# Autodesk Inventor assembly: ENSAMBLE GENERAL ACH-40L-2020-V
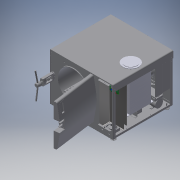
[picture p0: Inventor's stored thumbnail of the model, 180x180]
Saved by Autodesk Inventor 2017 (Build 210142000, 142)
## iProperties
Created: 2020-09-24
Part Number: ENSAMBLE GENERAL ACH-40L-2020-V
Description: STEP AP203
Document SubType Name: Assembly
Designer: USUARIO
Title: ENSAMBLE GENERAL ACH-40L-2020-V.STEP
Revision Number: ANY
Sending System: SolidWorks 2013
Preprocessor: SwSTEP 2.0
## Documents named in this file (42)
- D:\Laboratorio\Autoclave\Autoclave Horizontal\Sin Precamara\2020\Autoclave 40L con Vacio Insulab #0045883XX OP2020292\ENSAMBLE GENERAL ACH-40L-2020-V.iam
- D:\Laboratorio\Autoclave\Autoclave Horizontal\Sin Precamara\2020\Autoclave 40L con Vacio Insulab #0045883XX OP2020292\CUBIERTA FRONTAL ACH-40L-2020-V.ipt
- D:\Laboratorio\Autoclave\Autoclave Horizontal\Sin Precamara\2020\Autoclave 40L con Vacio Insulab #0045883XX OP2020292\BASE MUEBLE ACH-40L-2020-V.ipt
- D:\Laboratorio\Autoclave\Autoclave Horizontal\Sin Precamara\2020\Autoclave 40L con Vacio Insulab #0045883XX OP2020292\MARCO POSTERIOR ACH-40L-2020-V.ipt
- D:\Laboratorio\Autoclave\Autoclave Horizontal\Sin Precamara\2020\Autoclave 40L con Vacio Insulab #0045883XX OP2020292\ENSAMBLE TANQUE ACH-40L-2020-V.iam
- D:\Laboratorio\Autoclave\Autoclave Horizontal\Sin Precamara\2020\Autoclave 40L con Vacio Insulab #0045883XX OP2020292\ENSAMBLE PANEL FRONTAL ACH-40L-2020-V.iam
- D:\Laboratorio\Autoclave\Autoclave Horizontal\Sin Precamara\2020\Autoclave 40L con Vacio Insulab #0045883XX OP2020292\ENSAMBLE PUERTA ACH-40L-2020-V.iam
- D:\Laboratorio\Autoclave\Autoclave Horizontal\Sin Precamara\2020\Autoclave 40L con Vacio Insulab #0045883XX OP2020292\CAJA CONEXIONES ESPINAS ACH-40L-2020-V.ipt
- D:\Laboratorio\Autoclave\Autoclave Horizontal\Sin Precamara\2020\Autoclave 40L con Vacio Insulab #0045883XX OP2020292\PG-13,5.ipt
- D:\Laboratorio\Autoclave\Autoclave Horizontal\Sin Precamara\2020\Autoclave 40L con Vacio Insulab #0045883XX OP2020292\CAJA CONEXIONES ACH-40L-2020-V.ipt
- D:\Laboratorio\Autoclave\Autoclave Horizontal\Sin Precamara\2020\Autoclave 40L con Vacio Insulab #0045883XX OP2020292\REFUERZO INTERIOR ACH-40L-2020-V.ipt
- D:\Laboratorio\Autoclave\Autoclave Horizontal\Sin Precamara\2020\Autoclave 40L con Vacio Insulab #0045883XX OP2020292\VENTILADOR 9X9.ipt
- D:\Laboratorio\Autoclave\Autoclave Horizontal\Sin Precamara\2020\Autoclave 40L con Vacio Insulab #0045883XX OP2020292\ENSAMBLE GENERAL CIERRE JP2019-TTNR.iam
- D:\Laboratorio\Autoclave\Autoclave Horizontal\Sin Precamara\2020\Autoclave 40L con Vacio Insulab #0045883XX OP2020292\PIN CIERRE JP2019-TTNR.ipt
- D:\Laboratorio\Autoclave\Autoclave Horizontal\Sin Precamara\2020\Autoclave 40L con Vacio Insulab #0045883XX OP2020292\PIN BISAGRA JP2019-TTNR.ipt
- D:\Laboratorio\Autoclave\Autoclave Horizontal\Sin Precamara\2020\Autoclave 40L con Vacio Insulab #0045883XX OP2020292\PIVOTE CIERRE JP2019-TTNR.ipt
- D:\Laboratorio\Autoclave\Autoclave Horizontal\Sin Precamara\2020\Autoclave 40L con Vacio Insulab #0045883XX OP2020292\ENSAMBLE TAPA ACH-40L-2020-V.iam
- D:\Laboratorio\Autoclave\Autoclave Horizontal\Sin Precamara\2020\Autoclave 40L con Vacio Insulab #0045883XX OP2020292\ENSAMBLE RESERVORIO ACH-40L-2020-V.iam
- D:\Laboratorio\Autoclave\Autoclave Horizontal\Sin Precamara\2020\Autoclave 40L con Vacio Insulab #0045883XX OP2020292\CONTRATAPA SUPERIOR ACH-40L-2020-V.ipt
- D:\Laboratorio\Autoclave\Autoclave Horizontal\Sin Precamara\2020\Autoclave 40L con Vacio Insulab #0045883XX OP2020292\BANDEJA INTERIOR ACH-40L-2020-V.ipt
- D:\Laboratorio\Autoclave\Autoclave Horizontal\Sin Precamara\2020\Autoclave 40L con Vacio Insulab #0045883XX OP2020292\BOMBA DE VACIO THOMAS 2107CA20.ipt
- D:\Laboratorio\Autoclave\Autoclave Horizontal\Sin Precamara\2020\Autoclave 40L con Vacio Insulab #0045883XX OP2020292\CALDERIN ACH-40L-2020-V.ipt
- D:\Laboratorio\Autoclave\Autoclave Horizontal\Sin Precamara\2020\Autoclave 40L con Vacio Insulab #0045883XX OP2020292\CONTRATAPA INFERIOR ACH-40L-2020-V.ipt
- D:\Laboratorio\Autoclave\Autoclave Horizontal\Sin Precamara\2020\Autoclave 40L con Vacio Insulab #0045883XX OP2020292\CUBIERTA SUPERIOR ACH-40L-2020-V.ipt
- D:\Laboratorio\Autoclave\Autoclave Horizontal\Sin Precamara\2020\Autoclave 40L con Vacio Insulab #0045883XX OP2020292\CUBIERTA LATERAL ACH-40L-2020-V.ipt
- D:\Laboratorio\Autoclave\Autoclave Horizontal\Sin Precamara\2020\Autoclave 40L con Vacio Insulab #0045883XX OP2020292\ENSAMBLE RADIADOR ACH-40L-2020-V.iam
- D:\Laboratorio\Autoclave\Autoclave Horizontal\Sin Precamara\2020\Autoclave 40L con Vacio Insulab #0045883XX OP2020292\CUBIERTA LATERAL DERECHA ACH-40L-2020-V.ipt
- D:\Laboratorio\Autoclave\Autoclave Horizontal\Sin Precamara\2020\Autoclave 40L con Vacio Insulab #0045883XX OP2020292\CUBIERTA POSTERIOR ACH-40L-2020-V.ipt
- D:\Laboratorio\Autoclave\Autoclave Horizontal\Sin Precamara\2020\Autoclave 40L con Vacio Insulab #0045883XX OP2020292\ULKA EX5.ipt
- D:\Laboratorio\Autoclave\Autoclave Horizontal\Sin Precamara\2020\Autoclave 40L con Vacio Insulab #0045883XX OP2020292\DANFOSS EV215B.ipt
- D:\Laboratorio\Autoclave\Autoclave Horizontal\Sin Precamara\2020\Autoclave 40L con Vacio Insulab #0045883XX OP2020292\SOPORTE BOMBA AGUA ACH-40L-2020-V.ipt
- D:\Laboratorio\Autoclave\Autoclave Horizontal\Sin Precamara\2020\Autoclave 40L con Vacio Insulab #0045883XX OP2020292\SOPORTE VALVULAS ACH-40L-2020-V.ipt
- D:\Laboratorio\Autoclave\Autoclave Horizontal\Sin Precamara\2020\Autoclave 40L con Vacio Insulab #0045883XX OP2020292\PATA 5-16.ipt
- D:\Laboratorio\Autoclave\Autoclave Horizontal\Sin Precamara\2020\Autoclave 40L con Vacio Insulab #0045883XX OP2020292\VALVULA DE BOLA GENEBRE MH 3097-02 CW617N.ipt
- D:\Laboratorio\Autoclave\Autoclave Horizontal\Sin Precamara\2020\Autoclave 40L con Vacio Insulab #0045883XX OP2020292\ESPINAS DE PESCADO ACV-ACH.ipt
- D:\Laboratorio\Autoclave\Autoclave Horizontal\Sin Precamara\2020\Autoclave 40L con Vacio Insulab #0045883XX OP2020292\DERIVACION TANQUE ACH-40L-2020-V.ipt
- D:\Laboratorio\Autoclave\Autoclave Horizontal\Sin Precamara\2020\Autoclave 40L con Vacio Insulab #0045883XX OP2020292\TEE VALVULAS ACH-40L-2020-V.ipt
- D:\Laboratorio\Autoclave\Autoclave Horizontal\Sin Precamara\2020\Autoclave 40L con Vacio Insulab #0045883XX OP2020292\RESISTENCIA INTERIOR ACH-40L-2020-V.ipt
- D:\Laboratorio\Autoclave\Autoclave Horizontal\Sin Precamara\2020\Autoclave 40L con Vacio Insulab #0045883XX OP2020292\RESISTENCIA SECADO ACH-40L-2020-V.ipt
- D:\Laboratorio\Autoclave\Autoclave Horizontal\Sin Precamara\2020\Autoclave 40L con Vacio Insulab #0045883XX OP2020292\DEFLECTOR ACH-40L-2020-V.ipt
- D:\Laboratorio\Autoclave\Autoclave Horizontal\Sin Precamara\2020\Autoclave 40L con Vacio Insulab #0045883XX OP2020292\ACOPLE DEFLECTOR ACH-40L-2020-V.ipt
- D:\Laboratorio\Autoclave\Autoclave Horizontal\Sin Precamara\2020\Autoclave 40L con Vacio Insulab #0045883XX OP2020292\Schematic\Nextion Control SM\NextionControlV3.iam
## Components (52 placed, 52 different names)
1. CUBIERTA FRONTAL ACH-40L-2020-V_1
2. BASE MUEBLE ACH-40L-2020-V_2
3. MARCO POSTERIOR ACH-40L-2020-V_3
4. ENSAMBLE TANQUE ACH-40L-2020-V_4 [sub-assembly]
5. ENSAMBLE PANEL FRONTAL ACH-40L-2020-V_5 [sub-assembly]
6. ENSAMBLE PUERTA ACH-40L-2020-V_6 [sub-assembly]
7. CAJA CONEXIONES ESPINAS ACH-40L-2020-V_7
8. PG-13,5_8
9. CAJA CONEXIONES ACH-40L-2020-V_9 — Mate:1, Mate:2
10. REFUERZO INTERIOR ACH-40L-2020-V_10
11. REFUERZO INTERIOR ACH-40L-2020-V_11
12. VENTILADOR 9X9_12
13. ENSAMBLE GENERAL CIERRE JP2019-TTNR_13 [sub-assembly]
14. PIN CIERRE JP2019-TTNR_14
15. PIN BISAGRA JP2019-TTNR_15
16. PIN BISAGRA JP2019-TTNR_16
17. PIVOTE CIERRE JP2019-TTNR_17
18. ENSAMBLE TAPA ACH-40L-2020-V_18 [sub-assembly]
19. ENSAMBLE RESERVORIO ACH-40L-2020-V_19 [sub-assembly]
20. CONTRATAPA SUPERIOR ACH-40L-2020-V_20
21. BANDEJA INTERIOR ACH-40L-2020-V_21
22. BOMBA DE VACIO THOMAS 2107CA20_22
23. CALDERIN ACH-40L-2020-V_23
24. CONTRATAPA INFERIOR ACH-40L-2020-V_24
25. CUBIERTA SUPERIOR ACH-40L-2020-V_25
26. CUBIERTA LATERAL ACH-40L-2020-V_26
27. ENSAMBLE RADIADOR ACH-40L-2020-V_27 [sub-assembly]
28. CUBIERTA LATERAL DERECHA ACH-40L-2020-V_28
29. CUBIERTA POSTERIOR ACH-40L-2020-V_29
30. ULKA EX5_30
31. DANFOSS EV215B_31
32. SOPORTE BOMBA AGUA ACH-40L-2020-V_32
33. SOPORTE VALVULAS ACH-40L-2020-V_33
34. DANFOSS EV215B_34
35. DANFOSS EV215B_35
36. DANFOSS EV215B_36
37. DANFOSS EV215B_37
38. DANFOSS EV215B_38
39. PATA 5-16_39
40. PATA 5-16_40
41. PATA 5-16_41
42. PATA 5-16_42
43. PG-13,5_43
44. VALVULA DE BOLA GENEBRE MH 3097-02 CW617N_44
45. ESPINAS DE PESCADO ACV-ACH_45
46. DERIVACION TANQUE ACH-40L-2020-V_46
47. TEE VALVULAS ACH-40L-2020-V_47
48. RESISTENCIA INTERIOR ACH-40L-2020-V_48
49. RESISTENCIA SECADO ACH-40L-2020-V_49
50. DEFLECTOR ACH-40L-2020-V_50
51. ACOPLE DEFLECTOR ACH-40L-2020-V_51
52. NextionControlV3:1 [sub-assembly] — Mate:1, Mate:2
## Relationships (2: Mate 2)
- Mate:1 (10 mm): CAJA CONEXIONES ACH-40L-2020-V_9 ↔ NextionControlV3:1
- Mate:2 (20 mm): CAJA CONEXIONES ACH-40L-2020-V_9 ↔ NextionControlV3:1
